# Autodesk Inventor assembly: Mentor Ring
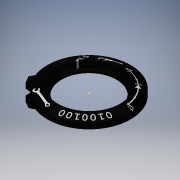
[picture p0: Inventor's stored thumbnail of the model, 180x180]
Saved by Autodesk Inventor 2016 (Build 200138000, 138)
## iProperties
Created: 2016-02-22
Part Number: Mentor Ring
Document SubType Name: Assembly
Designer: Spooner
Author: Spooner
## Documents named in this file (10)
- C:\Users\PLTW\Documents\Inventor\RoboCat Pin\Mentor Ring.iam
- C:\Users\PLTW\Documents\Inventor\RoboCat Pin\Mentor-Code ring.ipt
- C:\Users\PLTW\Documents\Inventor\RoboCat Pin\Mentor-Code text.ipt
- C:\Users\PLTW\Documents\Inventor\RoboCat Pin\Mentor-Mechanical ring.ipt
- C:\Users\PLTW\Documents\Inventor\RoboCat Pin\Mentor-Electrical ring.ipt
- C:\Users\PLTW\Documents\Inventor\RoboCat Pin\Mentor-Electrical text.ipt
- C:\Users\PLTW\Documents\Inventor\RoboCat Pin\Team Pin Mechanical-Left Wrench.ipt
- C:\Users\PLTW\Documents\Inventor\RoboCat Pin\Mentor-CAD ring.ipt
- C:\Users\PLTW\Documents\Inventor\RoboCat Pin\Mentor-CAD text.ipt
- C:\Users\PLTW\Documents\Inventor\RoboCat Pin\Team Pin Cad-Caliper.ipt
## Components (9 placed, 9 different names)
1. Mentor-Code ring:1 — Mate:1, Flush:1, Mate:2, Insert:1, Mate:3, Mate:7, Mate:8, Mate:9
2. Mentor-Code text:1 — Mate:7, Mate:8, Mate:9
3. Mentor-Mechanical ring:1 — Mate:1, Flush:1, Mate:2, Insert:2, Mate:4, Mate:10
4. Mentor-Electrical ring:1 — Insert:1, Mate:3, Mate:5, Mate:6, Insert:3
5. Mentor-Electrical text:1 — Mate:5, Mate:6
6. Team Pin Mechanical-Left Wrench:1 — Insert:2, Mate:4
7. Mentor-CAD ring:1 — Insert:3, Mate:10, Mate:11, Mate:12, Mate:13, Mate:14, Mate:15, Mate:16
8. Mentor-CAD text:1 — Mate:14, Mate:15, Mate:16
9. Team Pin Cad-Caliper:1 — Mate:11, Mate:12, Mate:13
## Relationships (20: Mate 16, Insert 3, Flush 1)
- Mate:1: Mentor-Code ring:1 ↔ Mentor-Mechanical ring:1
- Flush:1: Mentor-Code ring:1 ↔ Mentor-Mechanical ring:1
- Mate:2: Mentor-Code ring:1 ↔ Mentor-Mechanical ring:1
- Insert:1: Mentor-Code ring:1 ↔ Mentor-Electrical ring:1
- Mate:3: Mentor-Code ring:1 ↔ Mentor-Electrical ring:1
- Insert:2: Mentor-Mechanical ring:1 ↔ Team Pin Mechanical-Left Wrench:1
- Mate:4: Mentor-Mechanical ring:1 ↔ Team Pin Mechanical-Left Wrench:1
- Mate:5: Mentor-Electrical ring:1 ↔ Mentor-Electrical text:1
- Mate:6: Mentor-Electrical ring:1 ↔ Mentor-Electrical text:1
- Mate:7: Mentor-Code ring:1 ↔ Mentor-Code text:1
- Mate:8: Mentor-Code ring:1 ↔ Mentor-Code text:1
- Mate:9: Mentor-Code ring:1 ↔ Mentor-Code text:1
- Insert:3: Mentor-Electrical ring:1 ↔ Mentor-CAD ring:1
- Mate:10: Mentor-Mechanical ring:1 ↔ Mentor-CAD ring:1
- Mate:11: Mentor-CAD ring:1 ↔ Team Pin Cad-Caliper:1
- Mate:12: Mentor-CAD ring:1 ↔ Team Pin Cad-Caliper:1
- Mate:13: Mentor-CAD ring:1 ↔ Team Pin Cad-Caliper:1
- Mate:14: Mentor-CAD ring:1 ↔ Mentor-CAD text:1
- Mate:15: Mentor-CAD ring:1 ↔ Mentor-CAD text:1
- Mate:16: Mentor-CAD ring:1 ↔ Mentor-CAD text:1
